# Autodesk Inventor assembly: GY_521
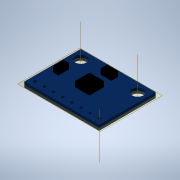
[picture p0: Inventor's stored thumbnail of the model, 180x180]
Saved by Autodesk Inventor 2021 (Build 250183000, 183)
## iProperties
Created: 2020-08-26
Part Number: GY_521
Material: Generisch
Document SubType Name: Assembly
Designer: ALEX
Mass: 0.607352 g
Surface Area: 12.0474 cm^2
Volume: 0.607352 cm^3
Density: 1 g/cm^3
Author: ALEX
## Documents named in this file (2)
- G:\Other computers\Mein Computer\TrainingConsol_220422\Workgroups\Workgroup\GY_521.iam
- G:\Other computers\Mein Computer\TrainingConsol_220422\Workgroups\Workgroup\GY_521.ipt
## Components (1 placed, 1 different names)
1. GY_521:1 — Passend:2
## Relationships (1: Mate 1)
- Passend:2 [Mate]: GY_521:1
